# Autodesk Inventor assembly: spool
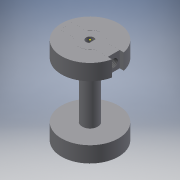
[picture p0: Inventor's stored thumbnail of the model, 180x180]
Saved by Autodesk Inventor 2017 (Build 210142000, 142)
## iProperties
Created: 2017-03-22
Part Number: spool
Document SubType Name: Assembly
Designer: s4371792
Author: s4371792
## Documents named in this file (4)
- E:\spool.iam
- E:\plate.ipt
- C:\Users\s4371792\Downloads\Stepper_Key.ipt
- E:\endPlate.ipt
## Components (3 placed, 3 different names)
1. plate:1 — Rigid:1
2. Stepper_Key:1 — Rigid:1, Rigid:2
3. endPlate:1 — Rigid:2
## Relationships (2: WeldJoint 2)
- Rigid:1 [WeldJoint]: plate:1 ↔ Stepper_Key:1
- Rigid:2 [WeldJoint] (-10 mm): Stepper_Key:1 ↔ endPlate:1
